# Autodesk Inventor assembly: DRO Case 3
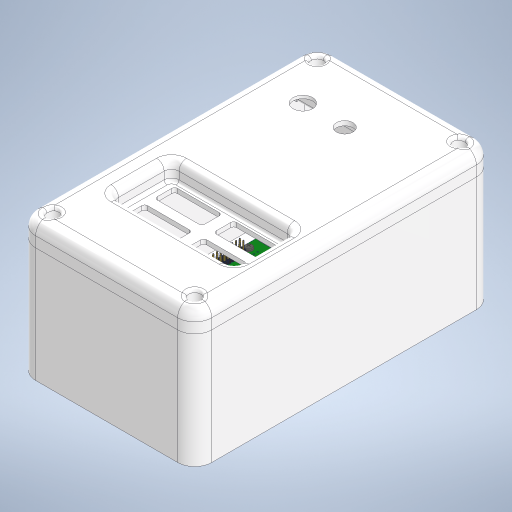
[picture p0: Inventor's stored thumbnail of the model, 512x512]
Saved by Autodesk Inventor 2024 (Build 280153000, 153)
## iProperties
Created: 2024-03-12
Part Number: DRO Case 3
Document SubType Name: Assembly
Designer: AdminForWorker
Title: DRO Case 3 v9
Author: AdminForWorker
## Documents named in this file (4)
- C:\Users\Stefano\Desktop\inventor-dro-case\DRO Case 3.iam
- C:\Users\Stefano\Desktop\inventor-dro-case\Component1.ipt
- C:\Users\Stefano\Desktop\inventor-dro-case\Component4.ipt
- C:\Users\Stefano\Desktop\inventor-dro-case\raspberry pi display.iam
## Components (3 placed, 3 different names)
1. Body — Rotational:1, Mate:1
2. Back Cover
3. raspberry pi display:1 [sub-assembly] — Rotational:1, Mate:1
## Relationships (2: RevoluteJoint 1, Mate 1)
- Rotational:1 [RevoluteJoint]: Body ↔ raspberry pi display:1
- Mate:1: Body ↔ raspberry pi display:1
